# Autodesk Inventor assembly: stemRibAssembly01
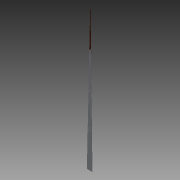
[picture p0: Inventor's stored thumbnail of the model, 180x180]
Saved by Autodesk Inventor 2013 (Build 170138000, 138)
## iProperties
Created: 2014-08-26
Part Number: stemRibAssembly01
Document SubType Name: Assembly
Designer: Nano
Author: Nano
## Documents named in this file (5)
- C:\Users\Nano\Documents\InventorByron\InventorMasterProject\octoBoto\stemRibAssembly01.iam
- C:\Users\Nano\Documents\InventorByron\InventorMasterProject\octoBoto\octoBotoStemRibSectA_V01.ipt
- C:\Users\Nano\Documents\InventorByron\InventorMasterProject\octoBoto\octoBotoStemRibSectB_v01.ipt
- C:\Users\Nano\Documents\InventorByron\InventorMasterProject\octoBoto\octoBotoStemSectC_v01.ipt
- C:\Users\Nano\Documents\InventorByron\InventorMasterProject\octoBoto\octoBotoStemSectD_v01.ipt
## Components (4 placed, 4 different names)
1. octoBotoStemRibSectA_V01:1 — Flush:1, Flush:2
2. octoBotoStemRibSectB_v01:1 — Flush:1, Flush:2, Flush:3, Flush:4
3. octoBotoStemSectC_v01:1 — Flush:3, Flush:4, Flush:5, Flush:6
4. octoBotoStemSectD_v01:1 — Flush:5, Flush:6
## Relationships (6: Flush 6)
- Flush:1: octoBotoStemRibSectA_V01:1 ↔ octoBotoStemRibSectB_v01:1
- Flush:2: octoBotoStemRibSectA_V01:1 ↔ octoBotoStemRibSectB_v01:1
- Flush:3: octoBotoStemRibSectB_v01:1 ↔ octoBotoStemSectC_v01:1
- Flush:4: octoBotoStemRibSectB_v01:1 ↔ octoBotoStemSectC_v01:1
- Flush:5: octoBotoStemSectC_v01:1 ↔ octoBotoStemSectD_v01:1
- Flush:6: octoBotoStemSectC_v01:1 ↔ octoBotoStemSectD_v01:1
